# Autodesk Inventor assembly: Interface assy
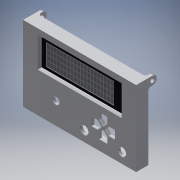
[picture p0: Inventor's stored thumbnail of the model, 180x180]
Saved by Autodesk Inventor 2018 (Build 220112000, 112)
## iProperties
Created: 2018-03-12
Part Number: Interface assy
Document SubType Name: Assembly
Designer: Gabriel Smolnycki
Author: Gabriel Smolnycki
## Documents named in this file (3)
- E:\Madog\planb\mechanics\Subassemblies\Interface assy.iam
- E:\Madog\planb\mechanics\Controls\Interface Frame.ipt
- E:\Madog\planb\mechanics\Electronics\NHD-0420CW.ipt
## Components (2 placed, 2 different names)
1. Interface Frame:1 — Mate:1, Mate:2, Mate:3
2. NHD-0420CW:1 — Mate:1, Mate:2, Mate:3
## Relationships (3: Mate 3)
- Mate:1 (0.25 mm): Interface Frame:1 ↔ NHD-0420CW:1
- Mate:2 (0.25 mm): Interface Frame:1 ↔ NHD-0420CW:1
- Mate:3 (2 mm): Interface Frame:1 ↔ NHD-0420CW:1
